# Autodesk Inventor assembly: Z-Y Axis Bracket
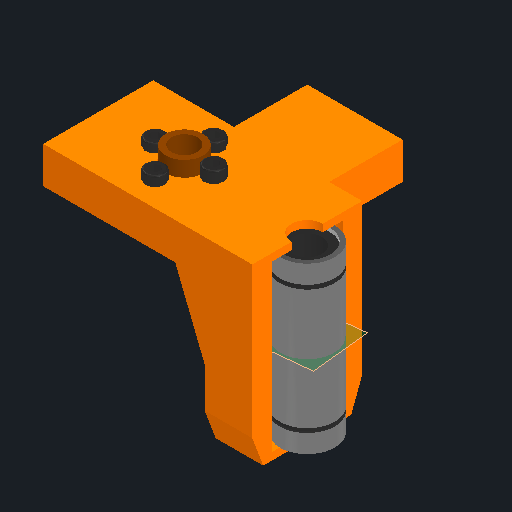
[picture p0: Inventor's stored thumbnail of the model, 512x512]
Saved by Autodesk Inventor 2025.1 (Build 291241000, 241)
## iProperties
Created: 2024-11-11
Part Number: Z-Y Axis Bracket
Document SubType Name: Assembly
Designer: jerem
Author: jerem
## Documents named in this file (5)
- C:\Users\jerem\Documents\GitHub\Perovskite-Automated-Synthesis-System\CAD\Gantry\Z-Y Axis Bracket.iam
- C:\Users\jerem\Documents\GitHub\Perovskite-Automated-Synthesis-System\CAD\Gantry\Z axis bracket.ipt
- C:\Users\jerem\Documents\GitHub\Perovskite-Automated-Synthesis-System\CAD\Non 3D Printed Parts\Leadscrew.ipt
- C:\Users\jerem\Documents\GitHub\Perovskite-Automated-Synthesis-System\CAD\Non 3D Printed Parts\Linear Rails\Linear Bearing 8mm Round.ipt
- C:\Users\jerem\Documents\GitHub\Perovskite-Automated-Synthesis-System\CAD\Non 3D Printed Parts\Screws\M3x12.ipt
## Components (7 placed, 4 different names)
1. Z axis bracket:1 — Mate:1, Mate:2, Mate:3, Mate:5, Mate:6, Mate:7, Mate:8, Mate:9, Mate:10
2. Leadscrew:1 — Mate:1, Mate:2, Mate:3
3. Linear Bearing 8mm Round:1 — Mate:5, Mate:6
4. M3x12:1 — Mate:7
5. M3x12:2 — Mate:8
6. M3x12:3 — Mate:9
7. M3x12:4 — Mate:10
## Relationships (9: Mate 9)
- Mate:1: Z axis bracket:1 ↔ Leadscrew:1
- Mate:2: Z axis bracket:1 ↔ Leadscrew:1
- Mate:3: Z axis bracket:1 ↔ Leadscrew:1
- Mate:5: Z axis bracket:1 ↔ Linear Bearing 8mm Round:1
- Mate:6: Z axis bracket:1 ↔ Linear Bearing 8mm Round:1
- Mate:7: Z axis bracket:1 ↔ M3x12:1
- Mate:8: Z axis bracket:1 ↔ M3x12:2
- Mate:9: Z axis bracket:1 ↔ M3x12:3
- Mate:10: Z axis bracket:1 ↔ M3x12:4
